# Autodesk Inventor assembly: ImpresionGarra
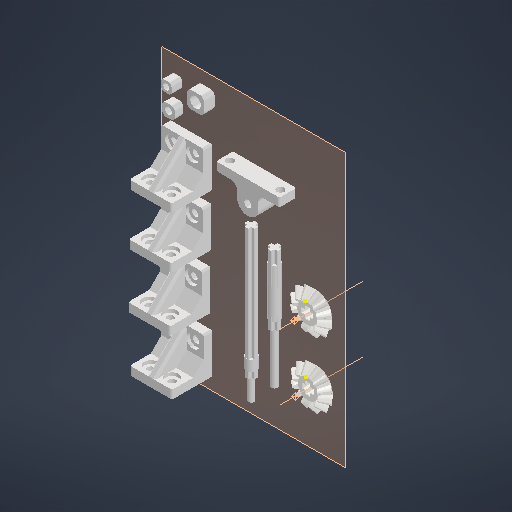
[picture p0: Inventor's stored thumbnail of the model, 512x512]
Saved by Autodesk Inventor 2026.3 (Build 303398000, 398)
## iProperties
Created: 2026-05-15
Part Number: ImpresionGarra
Document SubType Name: Assembly
Designer: Caro
Author: Caro
## Documents named in this file (9)
- C:\Users\Caro\JoseCarlos\TEC\TFG\Inventor\PiezasSTD\EnsamblesDeImpresion\ImpresionGarra.iam
- C:\Users\Caro\JoseCarlos\TEC\TFG\Inventor\PiezasSTD\TapónEje.ipt
- C:\Users\Caro\JoseCarlos\TEC\TFG\Inventor\PiezasSTD\T.ipt
- C:\Users\Caro\JoseCarlos\TEC\TFG\Inventor\PiezasSTD\SoporteEjes.ipt
- C:\Users\Caro\JoseCarlos\TEC\TFG\Inventor\PiezasSTD\ReyenedorTornillo3M.ipt
- C:\Users\Caro\JoseCarlos\TEC\TFG\Inventor\PiezasSTD\RetenedorEjeGarraVerticalSuperior.ipt
- C:\Users\Caro\JoseCarlos\TEC\TFG\Inventor\PiezasSTD\EjecilindroGarraSTD.ipt
- C:\Users\Caro\JoseCarlos\TEC\TFG\Inventor\PiezasSTD\EjeCilintroSuperiorGarra.ipt
- C:\Users\Caro\JoseCarlos\TEC\TFG\Inventor\PiezasSTD\EnsambleGarraSTD\Design Accelerator\Engranaje biselado11.ipt
## Components (12 placed, 8 different names)
1. TapónEje:1 — Coincidencia:1
2. T:1 — Coincidencia:2, Coincidencia:4
3. T:2 — Coincidencia:3
4. T:3 — Coincidencia:6
5. T:4 — Coincidencia:14
6. SoporteEjes:1 — Coincidencia:5
7. ReyenedorTornillo3M:1 — Coincidencia:7, Coincidencia:8
8. RetenedorEjeGarraVerticalSuperior:1 — Coincidencia:9
9. EjecilindroGarraSTD:1 — Coincidencia:10
10. EjeCilintroSuperiorGarra:1 — Coincidencia:11
11. Engranaje biselado1:1 — Coincidencia:12
12. Engranaje biselado1:2 — Coincidencia:13
## Relationships (14: Mate 14)
- Coincidencia:1 [Mate]: TapónEje:1
- Coincidencia:2 [Mate]: T:1
- Coincidencia:3 [Mate]: T:2
- Coincidencia:4 [Mate]: T:1
- Coincidencia:5 [Mate]: SoporteEjes:1
- Coincidencia:6 [Mate]: T:3
- Coincidencia:7 [Mate]: ReyenedorTornillo3M:1
- Coincidencia:8 [Mate]: ReyenedorTornillo3M:1
- Coincidencia:9 [Mate]: RetenedorEjeGarraVerticalSuperior:1
- Coincidencia:10 [Mate]: EjecilindroGarraSTD:1
- Coincidencia:11 [Mate]: EjeCilintroSuperiorGarra:1
- Coincidencia:12 [Mate]: Engranaje biselado1:1
- Coincidencia:13 [Mate]: Engranaje biselado1:2
- Coincidencia:14 [Mate]: T:4
